# Autodesk Inventor assembly: Weapon (Weapon-Side Pulley)
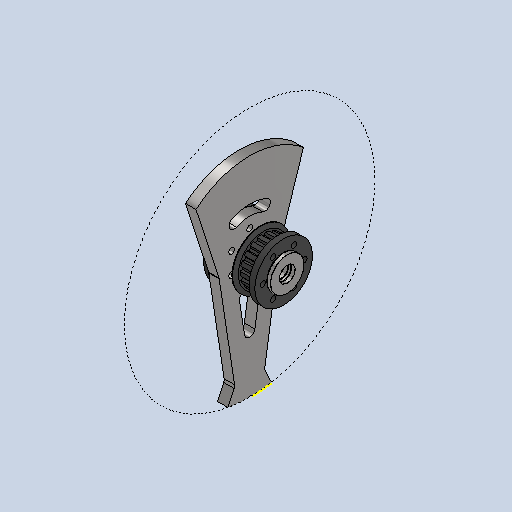
[picture p0: Inventor's stored thumbnail of the model, 512x512]
Saved by Autodesk Inventor 2023.2 (Build 272271000, 271)
## iProperties
Created: 2022-05-08
Part Number: Weapon (Weapon-Side Pulley)
Document SubType Name: Assembly
Designer: NCai2
Mass: 278.888 g
Surface Area: 324.19 cm^2
Volume: 48.7737 cm^3
Density: 5.718 g/cm^3
Author: NCai2
## Documents named in this file (7)
- E:\Documents\Inventor\Law - V1.0\Vertical Weapon Assembly (Type A)\Weapon (Weapon-Side Pulley).iam
- E:\Documents\Inventor\Law - V1.0\Vertical Weapon Assembly (Type A)\Thrust Ball Bearing.ipt
- E:\Documents\Inventor\Law - V1.0\Vertical Weapon Assembly (Type A)\5905K132_Needle-Roller Bearing.ipt
- E:\Documents\Inventor\Law - V1.0\Vertical Weapon Assembly (Type A)\Spacer 3-8x .125.ipt
- E:\Documents\Inventor\Law - V1.0\Vertical Weapon Assembly (Type A)\Blade (Bar 2).ipt
- E:\Documents\Inventor\Law - V1.0\Vertical Weapon Assembly (Type A)\XL Pulley 18T .25in Wd.ipt
- E:\Documents\Inventor\Law - V1.0\Vertical Weapon Assembly (Type A)\Blade (Bar 3).ipt
## Components (8 placed, 6 different names)
1. 5905K132_Needle-Roller Bearing:3 — Mate:12, Mate:14, Mate:15, Mate:18, Mate:31
2. 5905K132_Needle-Roller Bearing:4 — Mate:9, Mate:13, Mate:15, Mate:17, Mate:31
3. Thrust Ball Bearing:3 — Mate:9, Mate:16, Mate:17
4. Thrust Ball Bearing:4 — Mate:12, Mate:14, Mate:16, Mate:21, Mate:28, Mate:33
5. Blade (Bar 2):1 — Mate:13, Mate:19, Mate:20, Mate:29, Mate:30
6. Spacer 3-8x .125:1 — Mate:18, Mate:19, Mate:20, Mate:21, Mate:32, Mate:34
7. XL Pulley 18T .25in Wd:1 — Mate:28, Mate:29, Mate:30
8. Blade (Bar 3):1 — Mate:32, Mate:33, Mate:34
## Relationships (18: Mate 18)
- Mate:9: 5905K132_Needle-Roller Bearing:4 ↔ Thrust Ball Bearing:3
- Mate:12: 5905K132_Needle-Roller Bearing:3 ↔ Thrust Ball Bearing:4
- Mate:13: 5905K132_Needle-Roller Bearing:4 ↔ Blade (Bar 2):1
- Mate:14: 5905K132_Needle-Roller Bearing:3 ↔ Thrust Ball Bearing:4
- Mate:15: 5905K132_Needle-Roller Bearing:3 ↔ 5905K132_Needle-Roller Bearing:4
- Mate:16 (-38.1 mm): Thrust Ball Bearing:3 ↔ Thrust Ball Bearing:4
- Mate:17: 5905K132_Needle-Roller Bearing:4 ↔ Thrust Ball Bearing:3
- Mate:18: 5905K132_Needle-Roller Bearing:3 ↔ Spacer 3-8x .125:1
- Mate:19: Blade (Bar 2):1 ↔ Spacer 3-8x .125:1
- Mate:20: Blade (Bar 2):1 ↔ Spacer 3-8x .125:1
- Mate:21: Thrust Ball Bearing:4 ↔ Spacer 3-8x .125:1
- Mate:28 (-34.925 mm): Thrust Ball Bearing:4 ↔ XL Pulley 18T .25in Wd:1
- Mate:29: Blade (Bar 2):1 ↔ XL Pulley 18T .25in Wd:1
- Mate:30: Blade (Bar 2):1 ↔ XL Pulley 18T .25in Wd:1
- Mate:31: 5905K132_Needle-Roller Bearing:3 ↔ 5905K132_Needle-Roller Bearing:4
- Mate:32: Spacer 3-8x .125:1 ↔ Blade (Bar 3):1
- Mate:33: Thrust Ball Bearing:4 ↔ Blade (Bar 3):1
- Mate:34: Spacer 3-8x .125:1 ↔ Blade (Bar 3):1
